# Autodesk Inventor assembly: AtwoodsAsmy
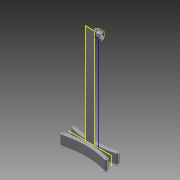
[picture p0: Inventor's stored thumbnail of the model, 180x180]
Saved by Autodesk Inventor 2012 (Build 160160000, 160)
## iProperties
Created: 2013-07-07
Part Number: AtwoodsAsmy
Document SubType Name: Assembly
Designer: 1
Author: 1
## Documents named in this file (5)
- D:\p3_metod1580library\figures\sources\M1-AtwoodsMachine\AtwoodsAsmy.iam
- D:\p3_metod1580library\figures\sources\M1-AtwoodsMachine\Atwoods-BaseBent.ipt
- D:\p3_metod1580library\figures\sources\M1-AtwoodsMachine\AdjLegStand.ipt
- D:\p3_metod1580library\figures\sources\M1-AtwoodsMachine\Ruler.ipt
- D:\p3_metod1580library\figures\sources\M1-AtwoodsMachine\BallHolder.ipt
## Components (8 placed, 4 different names)
1. Atwoods-BaseBent:1 — Mate:1, Flush:1, Flush:2, Mate:2, Insert:3, Flush:3
2. Atwoods-BaseBent:2 — Mate:1, Flush:1, Flush:2, Insert:1, Insert:2
3. AdjLegStand:1 — Mate:2
4. AdjLegStand:2 — Insert:1
5. AdjLegStand:3 — Insert:2
6. AdjLegStand:4 — Insert:3
7. Ruler:1 — Flush:3, Mate:3, Mate:4, Flush:4, Flush:5
8. BallHolder:1 — Mate:3, Mate:4, Flush:4, Flush:5
## Relationships (12: Flush 5, Mate 4, Insert 3)
- Mate:1: Atwoods-BaseBent:1 ↔ Atwoods-BaseBent:2
- Flush:1: Atwoods-BaseBent:1 ↔ Atwoods-BaseBent:2
- Flush:2: Atwoods-BaseBent:1 ↔ Atwoods-BaseBent:2
- Mate:2: Atwoods-BaseBent:1 ↔ AdjLegStand:1
- Insert:1: Atwoods-BaseBent:2 ↔ AdjLegStand:2
- Insert:2: Atwoods-BaseBent:2 ↔ AdjLegStand:3
- Insert:3: Atwoods-BaseBent:1 ↔ AdjLegStand:4
- Flush:3: Atwoods-BaseBent:1 ↔ Ruler:1
- Mate:3: Ruler:1 ↔ BallHolder:1
- Mate:4: Ruler:1 ↔ BallHolder:1
- Flush:4: Ruler:1 ↔ BallHolder:1
- Flush:5 (10 mm): Ruler:1 ↔ BallHolder:1
